# Autodesk Inventor assembly: Chassis
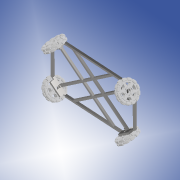
[picture p0: Inventor's stored thumbnail of the model, 180x180]
Saved by Autodesk Inventor 2017 (Build 210142000, 142)
## iProperties
Created: 2017-06-13
Part Number: Chassis
Document SubType Name: Assembly
Designer: zallen
Mass: 2949.64 g
Surface Area: 1083.98 cm^2
Volume: 375.75 cm^3
Density: 7.85 g/cm^3
Author: zallen
## Documents named in this file (7)
- C:\Users\zallen\Documents\GitHub\cr-laundry-robot\src\Base 2\Chassis\Chassis.iam
- C:\Users\zallen\Documents\GitHub\cr-laundry-robot\src\Base 2\Chassis\C001.ipt
- C:\Users\zallen\Documents\GitHub\cr-laundry-robot\src\Base 2\Chassis\C002.ipt
- C:\Users\zallen\Documents\GitHub\cr-laundry-robot\src\Base 2\Chassis\C003.ipt
- C:\Users\zallen\Documents\GitHub\cr-laundry-robot\src\Base 2\Chassis\C004.ipt
- C:\Users\zallen\Documents\GitHub\cr-laundry-robot\src\Base 2\Chassis\C005.ipt
- C:\Users\zallen\Documents\GitHub\cr-laundry-robot\src\Base 2\Chassis\217-2585.ipt
## Components (20 placed, 6 different names)
1. C001:1 — Mate:2, Mate:3, Mate:10, Mate:11, Mate:20, Mate:24
2. C001:2 — Mate:4, Mate:5, Mate:12, Mate:13, Mate:18, Mate:23
3. C002:1 — Mate:2, Mate:3, Mate:6, Mate:7, Mate:22, Mate:44
4. C002:2 — Mate:4, Mate:5, Mate:8, Mate:9, Mate:25, Mate:46
5. C003:1 — Mate:6, Mate:7, Mate:8, Mate:9
6. C002:3 — Mate:10, Mate:11, Mate:15, Mate:16, Mate:19, Mate:39
7. C002:4 — Mate:12, Mate:13, Mate:14, Mate:17, Mate:21, Mate:41
8. C003:2 — Mate:14, Mate:15, Mate:16, Mate:17
9. C004:1 — Mate:18, Mate:19, Mate:37, Mate:38
10. C004:2 — Mate:20, Mate:21, Mate:42
11. C004:3 — Mate:22, Mate:23, Mate:45
12. C004:4 — Mate:24, Mate:25, Mate:47
13. C005:1 — Mate:31, Mate:37, Mate:38, Mate:39, Mate:40
14. 217-2585:1 — Mate:31, Mate:40
15. C005:2 — Mate:41, Mate:42, Mate:43
16. 217-2585:2 — Mate:43
17. C005:3 — Mate:44, Mate:45, Mate:50, Mate:51
18. C005:4 — Mate:46, Mate:47, Mate:48, Mate:49
19. 217-2585:3 — Mate:48, Mate:49
20. 217-2585:4 — Mate:50, Mate:51
## Relationships (41: Mate 41)
- Mate:2: C001:1 ↔ C002:1
- Mate:3: C001:1 ↔ C002:1
- Mate:4: C001:2 ↔ C002:2
- Mate:5: C001:2 ↔ C002:2
- Mate:6: C002:1 ↔ C003:1
- Mate:7: C002:1 ↔ C003:1
- Mate:8: C002:2 ↔ C003:1
- Mate:9: C002:2 ↔ C003:1
- Mate:10: C001:1 ↔ C002:3
- Mate:11: C001:1 ↔ C002:3
- Mate:12: C001:2 ↔ C002:4
- Mate:13: C001:2 ↔ C002:4
- Mate:14: C002:4 ↔ C003:2
- Mate:15: C002:3 ↔ C003:2
- Mate:16: C002:3 ↔ C003:2
- Mate:17: C002:4 ↔ C003:2
- Mate:18: C001:2 ↔ C004:1
- Mate:19: C002:3 ↔ C004:1
- Mate:20: C001:1 ↔ C004:2
- Mate:21: C002:4 ↔ C004:2
- Mate:22: C002:1 ↔ C004:3
- Mate:23: C001:2 ↔ C004:3
- Mate:24: C001:1 ↔ C004:4
- Mate:25: C002:2 ↔ C004:4
- Mate:31: C005:1 ↔ 217-2585:1
- [Mate]: C005:2 ↔ 217-2585:2
- Mate:37: C004:1 ↔ C005:1
- Mate:38: C004:1 ↔ C005:1
- Mate:39: C002:3 ↔ C005:1
- Mate:40: C005:1 ↔ 217-2585:1
- Mate:41: C002:4 ↔ C005:2
- Mate:42: C004:2 ↔ C005:2
- Mate:43: C005:2 ↔ 217-2585:2
- Mate:44: C002:1 ↔ C005:3
- Mate:45: C004:3 ↔ C005:3
- Mate:46: C002:2 ↔ C005:4
- Mate:47: C004:4 ↔ C005:4
- Mate:48: C005:4 ↔ 217-2585:3
- Mate:49: C005:4 ↔ 217-2585:3
- Mate:50: C005:3 ↔ 217-2585:4
- Mate:51: C005:3 ↔ 217-2585:4
## Named parameters: d36_d33 = 0 mm
